# Autodesk Inventor assembly: ASY ДМФ 040 кольцо под шпильки КОРМА
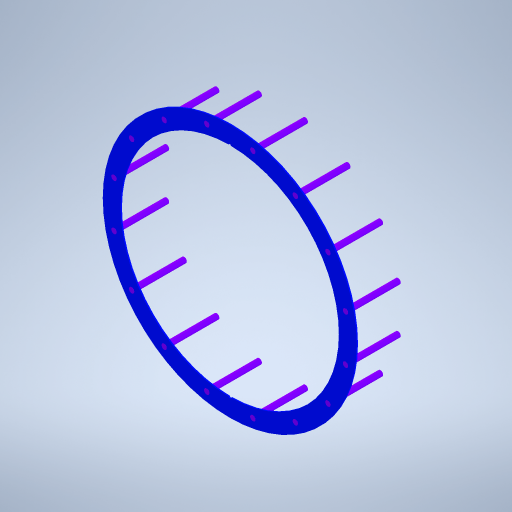
[picture p0: Inventor's stored thumbnail of the model, 512x512]
Saved by Autodesk Inventor 2024.2 (Build 282272000, 272)
## iProperties
Created: 2024-05-08
Part Number: ASY ДМФ 040 кольцо под шпильки КОРМА
Document SubType Name: Assembly
Designer: pokla
Stock Number: ДМФ 040 кольцо под шпильки КОРМА
Author: pokla
## Documents named in this file (4)
- C:\Users\user\YandexDisk\домашниий пк\Inventor\DMF-Disk-Micro-Filter\ASY ДМФ 070 кольцо под шпильки КОРМА наружное.iam
- C:\Users\user\YandexDisk\домашниий пк\Inventor\DMF-Disk-Micro-Filter\ДМФ 041 кольцо под шпильки КОРМА.ipt
- C:\Users\user\YandexDisk\домашниий пк\Inventor\DMF-Disk-Micro-Filter\ДМФ 042 шпилька 1.ipt
- C:\Users\user\YandexDisk\домашниий пк\Inventor\DMF-Disk-Micro-Filter\ДМФ 000 размеры.ipt
## Components (17 placed, 2 different names)
1. ДМС 011 кольцо под шпильки корма:1 — Rigid:1
2. ДМФ 042 шпилька 1:1 — Rigid:1
3. ДМФ 042 шпилька 1:2
4. ДМФ 042 шпилька 1:3
5. ДМФ 042 шпилька 1:4
6. ДМФ 042 шпилька 1:5
7. ДМФ 042 шпилька 1:6
8. ДМФ 042 шпилька 1:7
9. ДМФ 042 шпилька 1:8
10. ДМФ 042 шпилька 1:9
11. ДМФ 042 шпилька 1:10
12. ДМФ 042 шпилька 1:11
13. ДМФ 042 шпилька 1:12
14. ДМФ 042 шпилька 1:13
15. ДМФ 042 шпилька 1:14
16. ДМФ 042 шпилька 1:15
17. ДМФ 042 шпилька 1:16
## Component patterns: (16 elements, first: ДМФ 042 шпилька 1:1)
## Relationships (1: WeldJoint 1)
- Rigid:1 [WeldJoint]: ДМС 011 кольцо под шпильки корма:1 ↔ ДМФ 042 шпилька 1:1
